# Autodesk Inventor assembly: Gantry1
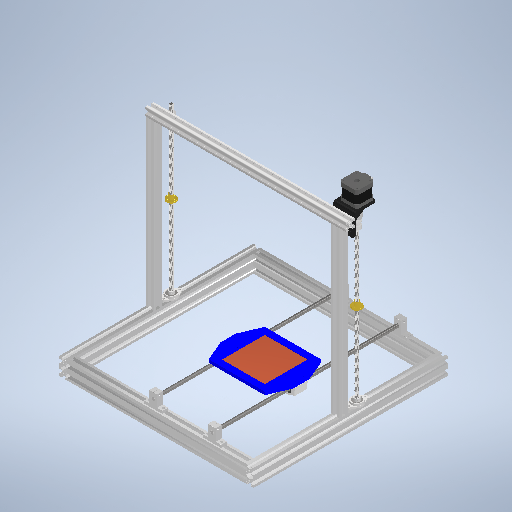
[picture p0: Inventor's stored thumbnail of the model, 512x512]
Saved by Autodesk Inventor 2025.2 (Build 292293000, 293)
## iProperties
Created: 2025-05-31
Part Number: Gantry1
Document SubType Name: Assembly
Designer: Simon
Author: Simon
## Documents named in this file (18)
- C:\Users\Simon\Projects\Hydrogel-3D-Printer\Hardware\Bioprinter Machine Design\Gantry Concept 1\Gantry1.iam
- C:\Users\Simon\Projects\Hydrogel-3D-Printer\Hardware\Bioprinter Machine Design\Gantry Concept 1\SteelShaft_444mm.ipt
- C:\Users\Simon\Projects\Hydrogel-3D-Printer\Hardware\Bioprinter Machine Design\PartsFolder\SK8_LinearShaftSupport.ipt
- C:\Users\Simon\Projects\Hydrogel-3D-Printer\Hardware\Bioprinter Machine Design\PartsFolder\PeltierTEC1_12706.ipt
- C:\Users\Simon\Projects\Hydrogel-3D-Printer\Hardware\Bioprinter Machine Design\PartsFolder\SC8UU\SC8UU.iam
- C:\Users\Simon\Projects\Hydrogel-3D-Printer\Hardware\Bioprinter Machine Design\Gantry Concept 1\BedPlate.ipt
- C:\Users\Simon\Projects\Hydrogel-3D-Printer\Hardware\Bioprinter Machine Design\Gantry Concept 1\BedHousingFrame.ipt
- C:\Users\Simon\Projects\Hydrogel-3D-Printer\Hardware\Bioprinter Machine Design\Gantry Concept 1\2040_AluminimProfile_450.ipt
- C:\Users\Simon\Projects\Hydrogel-3D-Printer\Hardware\Bioprinter Machine Design\Gantry Concept 1\2040_AluminimProfile_410.ipt
- C:\Users\Simon\Projects\Hydrogel-3D-Printer\Hardware\Bioprinter Machine Design\PartsFolder\bracket nema 17.ipt
- C:\Users\Simon\Projects\Hydrogel-3D-Printer\Hardware\Bioprinter Machine Design\Gantry Concept 1\2020_AluminiumProfile_380.ipt
- C:\Users\Simon\Projects\Hydrogel-3D-Printer\Hardware\Bioprinter Machine Design\PartsFolder\Pillow Block Bearing 1\Zinc Alloy Pillow Block Flange Bearing KFL08 ID-8mm.iam
- C:\Users\Simon\Projects\Hydrogel-3D-Printer\Hardware\Bioprinter Machine Design\Gantry Concept 1\TR8x8-4_LeadScrew_385mm.ipt
- C:\Users\Simon\Projects\Hydrogel-3D-Printer\Hardware\Bioprinter Machine Design\PartsFolder\Stepper_17HS4401.ipt
- C:\Users\Simon\Projects\Hydrogel-3D-Printer\Hardware\Bioprinter Machine Design\PartsFolder\GT2_20T_8.ipt
- C:\Users\Simon\Projects\Hydrogel-3D-Printer\Hardware\Bioprinter Machine Design\PartsFolder\Flexible Coupling 5,8.ipt
- C:\Users\Simon\Projects\Hydrogel-3D-Printer\Hardware\Bioprinter Machine Design\Gantry Concept 1\2020_AluminiumProfile_465.ipt
- C:\Users\Simon\Projects\Hydrogel-3D-Printer\Hardware\Bioprinter Machine Design\PartsFolder\TR8x8-4_Nut.ipt
## Components (29 placed, 17 different names)
1. SteelShaft_444mm:1 — Mate:1, Mate:3, Flush:1, Flush:4, Mate:5
2. SteelShaft_444mm:2 — Mate:2, Mate:4, Flush:2, Flush:3, Mate:6
3. SK8_LinearShaftSupport:1 — Mate:1, Flush:1, Flush:5, Flush:6, Mate:26
4. SK8_LinearShaftSupport:2 — Mate:2, Flush:2, Flush:5, Flush:6, Mate:23, Flush:19
5. SK8_LinearShaftSupport:3 — Mate:3, Flush:4, Mate:25
6. SK8_LinearShaftSupport:4 — Mate:4, Flush:3, Mate:24
7. PeltierTEC1_12706:1 — Mate:7, Flush:7, Flush:8
8. SC8UU:1 [sub-assembly] — Mate:5, Mate:11, Flush:9, Flush:11, Flush:12
9. SC8UU:2 [sub-assembly] — Mate:6, Flush:10, Mate:12, Flush:11
10. BedPlate:1 — Mate:7, Flush:7, Flush:8, Mate:8, Mate:9, Mate:10
11. BedHousingFrame:1 — Mate:8, Mate:9, Mate:10, Mate:11, Flush:9, Flush:10, Mate:12, Flush:12
12. 2040_AluminimProfile_450:1 — Mate:17, Flush:13, Flush:14, Mate:19, Flush:17, Flush:18, Mate:21, Mate:27, Flush:21, Mate:30, Mate:32
13. 2040_AluminimProfile_450:2 — Mate:18, Flush:15, Flush:16, Mate:23, Mate:24, Mate:28, Flush:20, Mate:29, Mate:31
14. 2040_AluminimProfile_410:1 — Mate:17, Flush:13, Flush:14, Mate:18, Flush:15, Flush:16, Mate:20, Mate:26, Flush:19
15. 2040_AluminimProfile_410:2 — Mate:19, Flush:17, Flush:18, Mate:22, Mate:25
16. bracket nema 17:1 — Mate:36, Mate:37, Mate:40, Angle:1
17. 2020_AluminiumProfile_380:1 — Mate:28, Flush:20, Flush:22
18. 2020_AluminiumProfile_380:2 — Mate:27, Flush:21, Flush:22, Mate:35, Flush:25, Flush:26
19. Zinc Alloy Pillow Block Flange Bearing KFL08 ID-8mm:1 [sub-assembly] — Mate:29, Mate:31, Flush:23, Mate:33, Flush:28
20. Zinc Alloy Pillow Block Flange Bearing KFL08 ID-8mm:2 [sub-assembly] — Mate:30, Mate:32, Flush:23, Mate:34
21. TR8x8-4_LeadScrew_385mm:1 — Mate:33, Flush:24, Mate:36, Mate:38, Flush:28, Mate:41, Mate:42, Mate:45
22. TR8x8-4_LeadScrew_385mm:2 — Mate:34, Flush:24, Mate:43, Mate:46
23. Stepper_17HS4401:1 — Mate:38, Mate:39, Flush:27, Mate:40, Mate:41, Angle:1
24. GT2_20T_8:1 — Mate:42, Flush:29, Mate:44
25. GT2_20T_8:2 — Mate:43, Flush:29
26. Flexible Coupling 5,8:1 — Mate:39, Flush:27, Mate:44
27. 2020_AluminiumProfile_465:1 — Mate:35, Flush:25, Flush:26, Mate:37
28. TR8x8-4_Nut:1 — Mate:45, Flush:30
29. TR8x8-4_Nut:2 — Mate:46, Flush:30
## Relationships (73: Mate 42, Flush 30, Angle 1)
- Mate:1: SteelShaft_444mm:1 ↔ SK8_LinearShaftSupport:1
- Mate:2: SteelShaft_444mm:2 ↔ SK8_LinearShaftSupport:2
- Mate:3: SteelShaft_444mm:1 ↔ SK8_LinearShaftSupport:3
- Mate:4: SteelShaft_444mm:2 ↔ SK8_LinearShaftSupport:4
- Flush:1: SteelShaft_444mm:1 ↔ SK8_LinearShaftSupport:1
- Flush:2: SteelShaft_444mm:2 ↔ SK8_LinearShaftSupport:2
- Flush:3: SteelShaft_444mm:2 ↔ SK8_LinearShaftSupport:4
- Flush:4: SteelShaft_444mm:1 ↔ SK8_LinearShaftSupport:3
- Flush:5: SK8_LinearShaftSupport:1 ↔ SK8_LinearShaftSupport:2
- Flush:6: SK8_LinearShaftSupport:1 ↔ SK8_LinearShaftSupport:2
- Mate:5: SteelShaft_444mm:1 ↔ SC8UU:1
- Mate:6: SteelShaft_444mm:2 ↔ SC8UU:2
- Mate:7: PeltierTEC1_12706:1 ↔ BedPlate:1
- Flush:7 (-30 mm): PeltierTEC1_12706:1 ↔ BedPlate:1
- Flush:8 (30 mm): PeltierTEC1_12706:1 ↔ BedPlate:1
- Mate:8: BedPlate:1 ↔ BedHousingFrame:1
- Mate:9: BedPlate:1 ↔ BedHousingFrame:1
- Mate:10: BedPlate:1 ↔ BedHousingFrame:1
- Mate:11: SC8UU:1 ↔ BedHousingFrame:1
- Flush:9: SC8UU:1 ↔ BedHousingFrame:1
- Flush:10: SC8UU:2 ↔ BedHousingFrame:1
- Mate:12: SC8UU:2 ↔ BedHousingFrame:1
- Flush:11: SC8UU:1 ↔ SC8UU:2
- Flush:12 (50 mm): SC8UU:1 ↔ BedHousingFrame:1
- Mate:17: 2040_AluminimProfile_450:1 ↔ 2040_AluminimProfile_410:1
- Flush:13: 2040_AluminimProfile_450:1 ↔ 2040_AluminimProfile_410:1
- Flush:14: 2040_AluminimProfile_450:1 ↔ 2040_AluminimProfile_410:1
- Mate:18: 2040_AluminimProfile_450:2 ↔ 2040_AluminimProfile_410:1
- Flush:15: 2040_AluminimProfile_450:2 ↔ 2040_AluminimProfile_410:1
- Flush:16: 2040_AluminimProfile_450:2 ↔ 2040_AluminimProfile_410:1
- Mate:19: 2040_AluminimProfile_450:1 ↔ 2040_AluminimProfile_410:2
- Flush:17: 2040_AluminimProfile_450:1 ↔ 2040_AluminimProfile_410:2
- Flush:18: 2040_AluminimProfile_450:1 ↔ 2040_AluminimProfile_410:2
- Mate:20: 2040_AluminimProfile_410:1
- Mate:21: 2040_AluminimProfile_450:1
- Mate:22: 2040_AluminimProfile_410:2
- Mate:23: SK8_LinearShaftSupport:2 ↔ 2040_AluminimProfile_450:2
- Mate:24: SK8_LinearShaftSupport:4 ↔ 2040_AluminimProfile_450:2
- Mate:25: SK8_LinearShaftSupport:3 ↔ 2040_AluminimProfile_410:2
- Mate:26: SK8_LinearShaftSupport:1 ↔ 2040_AluminimProfile_410:1
- Flush:19 (3 mm): SK8_LinearShaftSupport:2 ↔ 2040_AluminimProfile_410:1
- Mate:27: 2040_AluminimProfile_450:1 ↔ 2020_AluminiumProfile_380:2
- Mate:28: 2040_AluminimProfile_450:2 ↔ 2020_AluminiumProfile_380:1
- Flush:20: 2040_AluminimProfile_450:2 ↔ 2020_AluminiumProfile_380:1
- Flush:21: 2040_AluminimProfile_450:1 ↔ 2020_AluminiumProfile_380:2
- Flush:22: 2020_AluminiumProfile_380:1 ↔ 2020_AluminiumProfile_380:2
- Mate:29: 2040_AluminimProfile_450:2 ↔ Zinc Alloy Pillow Block Flange Bearing KFL08 ID-8mm:1
- Mate:30: 2040_AluminimProfile_450:1 ↔ Zinc Alloy Pillow Block Flange Bearing KFL08 ID-8mm:2
- Mate:31: 2040_AluminimProfile_450:2 ↔ Zinc Alloy Pillow Block Flange Bearing KFL08 ID-8mm:1
- Mate:32: 2040_AluminimProfile_450:1 ↔ Zinc Alloy Pillow Block Flange Bearing KFL08 ID-8mm:2
- Flush:23: Zinc Alloy Pillow Block Flange Bearing KFL08 ID-8mm:1 ↔ Zinc Alloy Pillow Block Flange Bearing KFL08 ID-8mm:2
- Mate:33: Zinc Alloy Pillow Block Flange Bearing KFL08 ID-8mm:1 ↔ TR8x8-4_LeadScrew_385mm:1
- Mate:34: Zinc Alloy Pillow Block Flange Bearing KFL08 ID-8mm:2 ↔ TR8x8-4_LeadScrew_385mm:2
- Flush:24: TR8x8-4_LeadScrew_385mm:1 ↔ TR8x8-4_LeadScrew_385mm:2
- Mate:35: 2020_AluminiumProfile_380:2 ↔ 2020_AluminiumProfile_465:1
- Flush:25: 2020_AluminiumProfile_380:2 ↔ 2020_AluminiumProfile_465:1
- Flush:26: 2020_AluminiumProfile_380:2 ↔ 2020_AluminiumProfile_465:1
- Mate:36: bracket nema 17:1 ↔ TR8x8-4_LeadScrew_385mm:1
- Mate:37: bracket nema 17:1 ↔ 2020_AluminiumProfile_465:1
- Mate:38: TR8x8-4_LeadScrew_385mm:1 ↔ Stepper_17HS4401:1
- Mate:39: Stepper_17HS4401:1 ↔ Flexible Coupling 5,8:1
- Flush:27 (5 mm): Stepper_17HS4401:1 ↔ Flexible Coupling 5,8:1
- Mate:40: bracket nema 17:1 ↔ Stepper_17HS4401:1
- Flush:28: Zinc Alloy Pillow Block Flange Bearing KFL08 ID-8mm:1 ↔ TR8x8-4_LeadScrew_385mm:1
- Mate:41: TR8x8-4_LeadScrew_385mm:1 ↔ Stepper_17HS4401:1
- Angle:1 (0 deg): bracket nema 17:1 ↔ Stepper_17HS4401:1
- Mate:42: TR8x8-4_LeadScrew_385mm:1 ↔ GT2_20T_8:1
- Mate:43: TR8x8-4_LeadScrew_385mm:2 ↔ GT2_20T_8:2
- Flush:29: GT2_20T_8:1 ↔ GT2_20T_8:2
- Mate:44 (5 mm): GT2_20T_8:1 ↔ Flexible Coupling 5,8:1
- Mate:45: TR8x8-4_LeadScrew_385mm:1 ↔ TR8x8-4_Nut:1
- Mate:46: TR8x8-4_LeadScrew_385mm:2 ↔ TR8x8-4_Nut:2
- Flush:30: TR8x8-4_Nut:1 ↔ TR8x8-4_Nut:2
